# Autodesk Inventor assembly: FE-00013
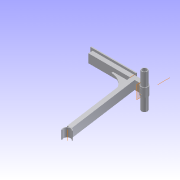
[picture p0: Inventor's stored thumbnail of the model, 180x180]
Saved by Autodesk Inventor 2012 (Build 160160000, 160)
## iProperties
Created: 2008-05-28
Part Number: FE-00013
Document SubType Name: Assembly
Designer: narosenberg
Description: Field Outrigger
Author: narosenberg
## Documents named in this file (9)
- C:\Data Folder\FRC 2012 Field\Components\FE-00013.iam
- C:\Data Folder\FRC 2012 Field\Components\FE-00013-06.ipt
- C:\Data Folder\FRC 2012 Field\Components\FE-00013-04.ipt
- C:\Data Folder\FRC 2012 Field\Components\FE-00013-02.ipt
- C:\Data Folder\FRC 2012 Field\Components\FE-00013-03.ipt
- C:\Data Folder\FRC 2012 Field\Components\FE-00013-05.ipt
- C:\Data Folder\FRC 2012 Field\Components\FE-00013-01.ipt
- C:\Data Folder\FRC 2012 Field\Components\FE-00013-07.ipt
- C:\Data Folder\FRC 2012 Field\Components\HW-00010.ipt
## Components (9 placed, 8 different names)
1. FE-00013-06:1 — Mate:1, Angle:1, Flush:1, Flush:2
2. FE-00013-04:1 — Mate:1, Angle:1, Flush:1, Flush:2, Tangent:1, Tangent:2, Flush:3, Angle:2, Mate:3, Flush:5, Flush:6, Mate:6, Flush:7
3. FE-00013-02:1 — Tangent:1, Tangent:2, Flush:3, Mate:2, Tangent:4, Insert:1, Mate:9, Mate:11, Mate:12, Tangent:6, Tangent:7
4. FE-00013-03:1 — Mate:3, Flush:6, Mate:5
5. FE-00013-05:1 — Mate:5, Mate:6, Flush:7, Tangent:3, Angle:3, Flush:8, Angle:6
6. FE-00013-01:1 — Tangent:3, Angle:3, Flush:8, Mate:7, Tangent:5, Angle:6
7. FE-00013-07:1 — Insert:1, Mate:8
8. HW-00010:1 — Mate:11, Tangent:6
9. HW-00010:2 — Mate:12, Tangent:7
## Relationships (31: Mate 11, Flush 7, Tangent 7, Angle 5, Insert 1)
- Mate:1: FE-00013-06:1 ↔ FE-00013-04:1
- Angle:1 (0 deg): FE-00013-06:1 ↔ FE-00013-04:1
- Flush:1 (12.7 mm): FE-00013-06:1 ↔ FE-00013-04:1
- Flush:2 (-12.7 mm): FE-00013-06:1 ↔ FE-00013-04:1
- Tangent:1: FE-00013-04:1 ↔ FE-00013-02:1
- Tangent:2: FE-00013-04:1 ↔ FE-00013-02:1
- Flush:3: FE-00013-04:1 ↔ FE-00013-02:1
- Mate:2: FE-00013-02:1
- Angle:2 (0 deg): FE-00013-04:1
- Mate:3: FE-00013-04:1 ↔ FE-00013-03:1
- Flush:5 (-247.65 mm): FE-00013-04:1
- Flush:6 (22.225 mm): FE-00013-04:1 ↔ FE-00013-03:1
- Mate:5: FE-00013-03:1 ↔ FE-00013-05:1
- Mate:6: FE-00013-04:1 ↔ FE-00013-05:1
- Flush:7: FE-00013-04:1 ↔ FE-00013-05:1
- Tangent:3: FE-00013-05:1 ↔ FE-00013-01:1
- Angle:3 (0 deg): FE-00013-05:1 ↔ FE-00013-01:1
- Flush:8: FE-00013-05:1 ↔ FE-00013-01:1
- Mate:7: FE-00013-01:1
- Angle:5 (0 deg)
- Tangent:4: FE-00013-02:1
- Tangent:5: FE-00013-01:1
- Insert:1 (-76.2 mm): FE-00013-02:1 ↔ FE-00013-07:1
- Mate:8: FE-00013-07:1
- Mate:9: FE-00013-02:1
- Mate:10
- Mate:11: FE-00013-02:1 ↔ HW-00010:1
- Mate:12: FE-00013-02:1 ↔ HW-00010:2
- Tangent:6: FE-00013-02:1 ↔ HW-00010:1
- Tangent:7: FE-00013-02:1 ↔ HW-00010:2
- Angle:6 (-27 deg): FE-00013-05:1 ↔ FE-00013-01:1
